# Autodesk Inventor assembly: 200-02-ROCKER-CONNECTOR-ASM-L
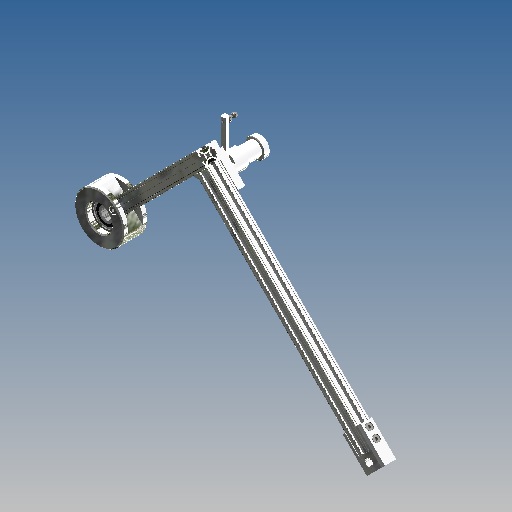
[picture p0: Inventor's stored thumbnail of the model, 512x512]
Saved by Autodesk Inventor 2018.2 (Build 222227000, 227)
## iProperties
Manager: feesmrt
Company: FRANCOR
Created: 2017-12-19
Part Number: 200-02-ROCKER-CONNECTOR-ASM-L
Project: Rescue Robot
Cost Center: -
Material: Generisch
Document SubType Name: Assembly
Designer: feesmrt
Engineer: feesmrt
Authority: feesmrt
Description: Rocker Connector Left Side ASM
Stock Number: 200-02-ROCKER-CONNECTOR-ASM-L
Subject: Rescue Robot
Author: feesmrt
Revision Number: 1
Title: Rocker Connector Left Side ASM
## Documents named in this file (6)
- D:\Programmierung\FRANC0R\CAD\02-Rocker-Bogie-Robot\200-ROCKER-BOGIE\200-02-ROCKER-CONNECTOR-ASM-L.iam
- D:\Programmierung\FRANC0R\CAD\02-Rocker-Bogie-Robot\200-ROCKER-BOGIE\200-20-ROCKER-CONNECTOR\200-20-ROCKER-CONNECTOR-ASM-01.iam
- D:\Programmierung\FRANC0R\CAD\02-Rocker-Bogie-Robot\900-COMPONENTS\900-50-PROFILES\90-50-PROFILES-30x30x250.ipt
- D:\Programmierung\FRANC0R\CAD\02-Rocker-Bogie-Robot\200-ROCKER-BOGIE\200-30-BOGIE-BEARING\200-30-BOGIE-BEARING-ASM-01.iam
- D:\Programmierung\FRANC0R\CAD\02-Rocker-Bogie-Robot\200-ROCKER-BOGIE\200-50-WHEEL-CONNECTOR\200-50-WHEEL-CONNECTOR-30MM-ASM-01.iam
- D:\Programmierung\FRANC0R\CAD\02-Rocker-Bogie-Robot\900-COMPONENTS\900-50-PROFILES\90-50-PROFILES-30x30x470.ipt
## Components (5 placed, 5 different names)
1. 200-20-ROCKER-CONNECTOR-ASM-01:1 [sub-assembly] — Passend:9, Fluchtend:3, Fluchtend:4, Fluchtend:5, Passend:11
2. 90-50-PROFILES-30x30x250:1 — Passend:5, Passend:6, Fluchtend:1, Passend:9, Fluchtend:3, Fluchtend:4, Passend:10
3. 200-30-BOGIE-BEARING-ASM-01:1 [sub-assembly] — Passend:5, Passend:6, Fluchtend:1
4. 200-50-WHEEL-CONNECTOR-30MM-ASM-01:1 [sub-assembly] — Passend:12, Fluchtend:6, Passend:13
5. 90-50-PROFILES-30x30x470:1 — Passend:10, Fluchtend:5, Passend:11, Passend:12, Fluchtend:6, Passend:13
## Relationships (12: Mate 7, Flush 5)
- Passend:5 [Mate]: 90-50-PROFILES-30x30x250:1 ↔ 200-30-BOGIE-BEARING-ASM-01:1
- Passend:6 [Mate]: 90-50-PROFILES-30x30x250:1 ↔ 200-30-BOGIE-BEARING-ASM-01:1
- Fluchtend:1 [Flush]: 90-50-PROFILES-30x30x250:1 ↔ 200-30-BOGIE-BEARING-ASM-01:1
- Passend:9 [Mate]: 200-20-ROCKER-CONNECTOR-ASM-01:1 ↔ 90-50-PROFILES-30x30x250:1
- Fluchtend:3 [Flush]: 200-20-ROCKER-CONNECTOR-ASM-01:1 ↔ 90-50-PROFILES-30x30x250:1
- Fluchtend:4 [Flush]: 200-20-ROCKER-CONNECTOR-ASM-01:1 ↔ 90-50-PROFILES-30x30x250:1
- Passend:10 [Mate]: 90-50-PROFILES-30x30x250:1 ↔ 90-50-PROFILES-30x30x470:1
- Fluchtend:5 [Flush]: 200-20-ROCKER-CONNECTOR-ASM-01:1 ↔ 90-50-PROFILES-30x30x470:1
- Passend:11 [Mate]: 200-20-ROCKER-CONNECTOR-ASM-01:1 ↔ 90-50-PROFILES-30x30x470:1
- Passend:12 [Mate]: 200-50-WHEEL-CONNECTOR-30MM-ASM-01:1 ↔ 90-50-PROFILES-30x30x470:1
- Fluchtend:6 [Flush]: 200-50-WHEEL-CONNECTOR-30MM-ASM-01:1 ↔ 90-50-PROFILES-30x30x470:1
- Passend:13 [Mate]: 200-50-WHEEL-CONNECTOR-30MM-ASM-01:1 ↔ 90-50-PROFILES-30x30x470:1
